# Autodesk Inventor assembly: Y_rail_Assembly_Rev3
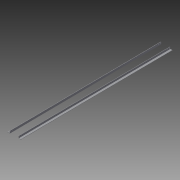
[picture p0: Inventor's stored thumbnail of the model, 180x180]
Saved by Autodesk Inventor 2015 (Build 190159000, 159)
## iProperties
Created: 2017-01-11
Part Number: Y_rail_Assembly_Rev3
Document SubType Name: Assembly
Designer: Guy
Mass: 1796.89 g
Surface Area: 4829.55 cm^2
Volume: 1200.62 cm^3
Density: 1.49664 g/cm^3
Author: Guy
## Documents named in this file (2)
- C:\Users\Ernest\Documents\Capstone-Project\doc\CAD\LowLevel_Rev3\Y_rail_Assembly_Rev3.iam
- C:\Users\Ernest\Documents\Capstone-Project\doc\CAD\LowLevel_Rev3\Y_Rail-SquareBar-Rev3.ipt
## Components (2 placed, 1 different names)
1. Y_Rail-SquareBar-Rev3:1 — Mate:97, Mate:99, Mate:102
2. Y_Rail-SquareBar-Rev3:2 — Mate:97, Mate:99, Mate:102
## Relationships (3: Mate 3)
- Mate:97: Y_Rail-SquareBar-Rev3:1 ↔ Y_Rail-SquareBar-Rev3:2
- Mate:99 (97 mm): Y_Rail-SquareBar-Rev3:1 ↔ Y_Rail-SquareBar-Rev3:2
- Mate:102: Y_Rail-SquareBar-Rev3:1 ↔ Y_Rail-SquareBar-Rev3:2
